# Autodesk Inventor assembly: VentilatorGesamt
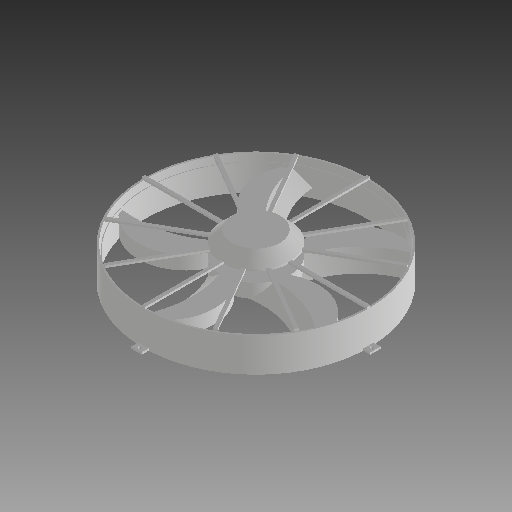
[picture p0: Inventor's stored thumbnail of the model, 512x512]
Saved by Autodesk Inventor 2021 (Build 250183000, 183)
## iProperties
Created: 2021-09-01
Part Number: VentilatorGesamt
Document SubType Name: Assembly
Designer: lukas
Stock Number: Ventilator
Author: lukas
## Documents named in this file (3)
- C:\Users\lukas\OneDrive - HTBLA Kaindorf\Diplomarbeit\Mechanik\InventorKonstruktion\VentilatorGesamt.iam
- C:\Users\lukas\OneDrive - HTBLA Kaindorf\Diplomarbeit\Mechanik\InventorKonstruktion\Ventilator2.ipt
- C:\Users\lukas\OneDrive - HTBLA Kaindorf\Diplomarbeit\Mechanik\InventorKonstruktion\Ventilator.ipt
## Components (2 placed, 2 different names)
1. Ventilator2:1 — Einfügen:1
2. Ventilator:1 — Einfügen:1
## Relationships (1: Insert 1)
- Einfügen:1 [Insert]: Ventilator2:1 ↔ Ventilator:1
